# Autodesk Inventor assembly: ARM 3 Real
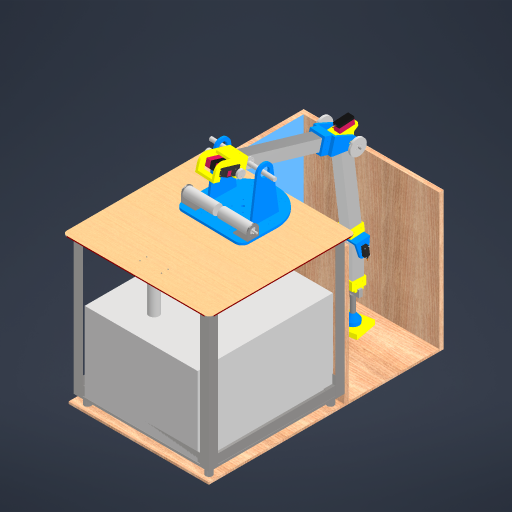
[picture p0: Inventor's stored thumbnail of the model, 512x512]
Saved by Autodesk Inventor 2023 (Build 270158000, 158)
## iProperties
Created: 2023-09-15
Part Number: ARM 3 Real
Document SubType Name: Assembly
Designer: Abhinav
Author: Abhinav
## Documents named in this file (7)
- C:\Users\Abhinav\Desktop\GRID\ARM 3\ARM 3 Real.iam
- C:\Users\Abhinav\Desktop\GRID\ARM 3\End-Effector\00_End-Effector.iam
- C:\Users\Abhinav\Desktop\GRID\ARM 3\End-Effector\End.ipt
- C:\Users\Abhinav\Desktop\GRID\ARM 3\Foundation\00_Foundation.iam
- C:\Users\Abhinav\Desktop\GRID\ARM 3\Foundation\Stage.ipt
- C:\Users\Abhinav\Desktop\GRID\ARM 3\Hand\00_Hand.iam
- C:\Users\Abhinav\Desktop\GRID\ARM 3\Forearm\00_Forearm.iam
## Components (6 placed, 6 different names)
1. 00_End-Effector:1 [sub-assembly] — Mate:6, Mate:7, Mate:8, Mate:9, Mate:10
2. End:1 — Mate:11, Mate:9, Mate:10
3. Stage:1 — Mate:1, Mate:2, Flush:1, Mate:11
4. 00_Foundation:1 [sub-assembly] — Mate:1, Mate:2, Flush:1, Mate:3, Flush:3
5. 00_Hand:1 [sub-assembly] — Mate:4, Mate:5, Mate:6, Mate:7, Mate:8
6. 00_Forearm:1 [sub-assembly] — Mate:3, Flush:3, Mate:4, Mate:5
## Relationships (13: Mate 11, Flush 2)
- Mate:1: Stage:1 ↔ 00_Foundation:1
- Mate:2: Stage:1 ↔ 00_Foundation:1
- Flush:1: Stage:1 ↔ 00_Foundation:1
- Mate:11: End:1 ↔ Stage:1
- Mate:3: 00_Foundation:1 ↔ 00_Forearm:1
- Flush:3 (-50 mm): 00_Foundation:1 ↔ 00_Forearm:1
- Mate:4: 00_Hand:1 ↔ 00_Forearm:1
- Mate:5 (15 mm): 00_Hand:1 ↔ 00_Forearm:1
- Mate:6: 00_End-Effector:1 ↔ 00_Hand:1
- Mate:7: 00_End-Effector:1 ↔ 00_Hand:1
- Mate:8: 00_End-Effector:1 ↔ 00_Hand:1
- Mate:9: 00_End-Effector:1 ↔ End:1
- Mate:10: 00_End-Effector:1 ↔ End:1
